# Autodesk Inventor assembly: hip_joint
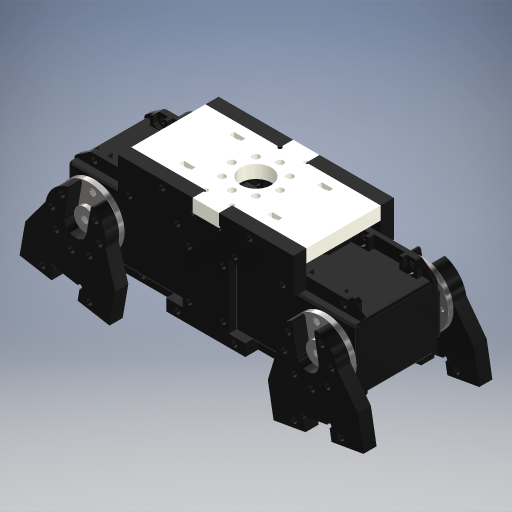
[picture p0: Inventor's stored thumbnail of the model, 512x512]
Saved by Autodesk Inventor 2024 (Build 280153000, 153)
## iProperties
Created: 2024-09-15
Part Number: hip_joint
Document SubType Name: Assembly
Designer: msi
Author: msi
## Documents named in this file (7)
- C:\Users\msi\GITHUB\19th_intern_kgh_fight_robot\부품\Lower_Body\Hip_joint\hip_joint.iam
- C:\Users\msi\GITHUB\19th_intern_kgh_fight_robot\부품\ROBOTIS(Inventor 2024 ver.)\다이나믹셀\MX-64T+idle.ipt.iam
- C:\Users\msi\GITHUB\19th_intern_kgh_fight_robot\부품\ROBOTIS(Inventor 2024 ver.)\혼\64-106Horn.ipt
- C:\Users\msi\GITHUB\19th_intern_kgh_fight_robot\부품\Lower_Body\Hip_joint\hip joint connection.ipt
- C:\Users\msi\GITHUB\19th_intern_kgh_fight_robot\부품\Lower_Body\Hip_joint\hip joint_body connection.ipt
- C:\Users\msi\GITHUB\19th_intern_kgh_fight_robot\부품\Lower_Body\Hip_joint\hip joint nad thigh connection_64.ipt
- MX-64T+idle.ipt
## Components (11 placed, 5 different names)
1. MX-64T+idle.ipt:1 [sub-assembly] — 삽입:6, 삽입:7, 삽입:8, 삽입:13, 삽입:14, 삽입:24, 각도:1
2. MX-64T+idle.ipt:2 [sub-assembly] — 삽입:5, 삽입:9, 삽입:10, 삽입:11, 삽입:12, 삽입:23, 각도:2
3. 64-106Horn:1 — 삽입:5, 삽입:19, 삽입:20
4. 64-106Horn:2 — 삽입:6, 삽입:21, 삽입:22
5. hip joint connection:1 — 삽입:7, 삽입:8, 삽입:9, 삽입:10, 삽입:17, 삽입:18
6. hip joint connection:2 — 삽입:11, 삽입:12, 삽입:13, 삽입:14, 삽입:15, 삽입:16
7. hip joint_body connection:1 — 삽입:15, 삽입:16, 삽입:17, 삽입:18
8. hip joint nad thigh connection_64:1 — 삽입:19, 삽입:20, 각도:2, 플러쉬:1
9. hip joint nad thigh connection_64:2 — 삽입:21, 삽입:22, 각도:1, 플러쉬:2
10. hip joint nad thigh connection_64:3 — 삽입:24, 플러쉬:2
11. hip joint nad thigh connection_64:4 — 삽입:23, 플러쉬:1
## Relationships (24: Insert 20, Angle 2, Flush 2)
- 삽입:5 [Insert]: MX-64T+idle.ipt:2 ↔ 64-106Horn:1
- 삽입:6 [Insert]: MX-64T+idle.ipt:1 ↔ 64-106Horn:2
- 삽입:7 [Insert]: MX-64T+idle.ipt:1 ↔ hip joint connection:1
- 삽입:8 [Insert]: MX-64T+idle.ipt:1 ↔ hip joint connection:1
- 삽입:9 [Insert]: MX-64T+idle.ipt:2 ↔ hip joint connection:1
- 삽입:10 [Insert]: MX-64T+idle.ipt:2 ↔ hip joint connection:1
- 삽입:11 [Insert]: MX-64T+idle.ipt:2 ↔ hip joint connection:2
- 삽입:12 [Insert]: MX-64T+idle.ipt:2 ↔ hip joint connection:2
- 삽입:13 [Insert]: MX-64T+idle.ipt:1 ↔ hip joint connection:2
- 삽입:14 [Insert]: MX-64T+idle.ipt:1 ↔ hip joint connection:2
- 삽입:15 [Insert]: hip joint connection:2 ↔ hip joint_body connection:1
- 삽입:16 [Insert]: hip joint connection:2 ↔ hip joint_body connection:1
- 삽입:17 [Insert]: hip joint connection:1 ↔ hip joint_body connection:1
- 삽입:18 [Insert]: hip joint connection:1 ↔ hip joint_body connection:1
- 삽입:19 [Insert]: 64-106Horn:1 ↔ hip joint nad thigh connection_64:1
- 삽입:20 [Insert]: 64-106Horn:1 ↔ hip joint nad thigh connection_64:1
- 삽입:21 [Insert]: 64-106Horn:2 ↔ hip joint nad thigh connection_64:2
- 삽입:22 [Insert]: 64-106Horn:2 ↔ hip joint nad thigh connection_64:2
- 삽입:23 [Insert]: MX-64T+idle.ipt:2 ↔ hip joint nad thigh connection_64:4
- 삽입:24 [Insert]: MX-64T+idle.ipt:1 ↔ hip joint nad thigh connection_64:3
- 각도:1 [Angle] (10 deg): MX-64T+idle.ipt:1 ↔ hip joint nad thigh connection_64:2
- 각도:2 [Angle] (-10 deg): MX-64T+idle.ipt:2 ↔ hip joint nad thigh connection_64:1
- 플러쉬:1 [Flush]: hip joint nad thigh connection_64:1 ↔ hip joint nad thigh connection_64:4
- 플러쉬:2 [Flush]: hip joint nad thigh connection_64:2 ↔ hip joint nad thigh connection_64:3
